# Autodesk Inventor assembly: MotorLeft
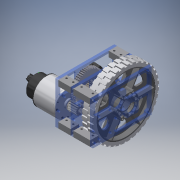
[picture p0: Inventor's stored thumbnail of the model, 180x180]
Saved by Autodesk Inventor 2019 (Build 230136000, 136)
## iProperties
Created: 2020-02-28
Part Number: MotorLeft
Document SubType Name: Assembly
Designer: james
Author: james
## Documents named in this file (13)
- F:\JimsRobot\FIRSTRobots\Design\TornadoPlatypus\MotorLeft.iam
- F:\JimsRobot\FIRSTRobots\Design\TornadoPlatypus\InsideMotorPlate.ipt
- F:\JimsRobot\FIRSTRobots\Design\Library\CTR\Falcon\217-6515 20191025.iam
- F:\JimsRobot\FIRSTRobots\Design\Library\CTR\Falcon\14T_20DP_FALCON.ipt
- F:\JimsRobot\FIRSTRobots\Design\Library\AndyMark\FR6ZZ Bearing.ipt
- F:\JimsRobot\FIRSTRobots\Design\TornadoPlatypus\MotorSpacerBlock.ipt
- F:\JimsRobot\FIRSTRobots\Design\Library\AndyMark\Toughbox d07.ipt
- F:\JimsRobot\FIRSTRobots\Design\Library\AndyMark\Toughbox d05.ipt
- F:\JimsRobot\FIRSTRobots\Design\Library\AndyMark\16t 20dp 375h with teeth.ipt
- F:\JimsRobot\FIRSTRobots\Design\Library\AndyMark\48t 20dp 500h with teeth.ipt
- F:\JimsRobot\FIRSTRobots\Design\Library\USDigital\E3-X-188-X-H-D-X.ipt
- F:\JimsRobot\FIRSTRobots\Design\Library\AndyMark\6 HiGrip Asm Rev II.iam
- F:\JimsRobot\FIRSTRobots\Design\TornadoPlatypus\MotorSpacerBlock2.ipt
## Components (19 placed, 12 different names)
1. InsideMotorPlate:1 — Mate:1, Mate:2, Mate:3, Mate:5, Mate:6, Mate:7, Mate:8, Mate:9, Mate:10, Mate:11, Flush:1, Mate:12, Flush:2, Mate:13, Flush:3, Mate:14, Flush:4, Mate:21, Mate:22, Mate:24
2. 217-6515 20191025:1 [sub-assembly] — Mate:1, Mate:2, Mate:3, Mate:4
3. 14T_20DP_FALCON:1 — Mate:4
4. FR6ZZ Bearing:1 — Mate:5, Mate:6, Mate:15, Flush:5, Mate:17
5. MotorSpacerBlock:1 — Mate:9, Mate:13, Flush:3, Mate:26, Mate:28
6. MotorSpacerBlock:2 — Mate:7, Mate:12, Flush:2
7. MotorSpacerBlock:3 — Mate:10, Mate:11, Flush:1
8. MotorSpacerBlock:4 — Mate:8, Mate:14, Flush:4, Mate:27
9. Toughbox d07:1 — Mate:15, Flush:5, Mate:16, Mate:19
10. Toughbox d05:1 — Mate:16, Mate:17, Mate:18, Mate:20
11. 16t 20dp 375h with teeth:1 — Mate:18, Mate:19
12. 48t 20dp 500h with teeth:1 — Mate:20, Mate:23
13. FR6ZZ Bearing:2 — Mate:21, Mate:22, Mate:23, Mate:25
14. E3-X-188-X-H-D-X:1 — Mate:24, Mate:25
15. InsideMotorPlate:2 — Mate:26, Mate:27, Mate:28, Mate:29, Mate:30, Mate:31, Mate:32, Mate:33, Flush:6, Mate:34, Flush:7
16. 6 HiGrip Asm Rev II:1 [sub-assembly] — Mate:29, Mate:30
17. MotorSpacerBlock2:1 — Mate:32, Mate:34, Flush:7, Mate:35, Mate:37
18. MotorSpacerBlock2:2 — Mate:31, Mate:33, Flush:6, Mate:36
19. InsideMotorPlate:3 — Mate:35, Mate:36, Mate:37
## Relationships (44: Mate 37, Flush 7)
- Mate:1: InsideMotorPlate:1 ↔ 217-6515 20191025:1
- Mate:2: InsideMotorPlate:1 ↔ 217-6515 20191025:1
- Mate:3: InsideMotorPlate:1 ↔ 217-6515 20191025:1
- Mate:4: 217-6515 20191025:1 ↔ 14T_20DP_FALCON:1
- Mate:5: InsideMotorPlate:1 ↔ FR6ZZ Bearing:1
- Mate:6: InsideMotorPlate:1 ↔ FR6ZZ Bearing:1
- Mate:7: InsideMotorPlate:1 ↔ MotorSpacerBlock:2
- Mate:8: InsideMotorPlate:1 ↔ MotorSpacerBlock:4
- Mate:9: InsideMotorPlate:1 ↔ MotorSpacerBlock:1
- Mate:10: InsideMotorPlate:1 ↔ MotorSpacerBlock:3
- Mate:11: InsideMotorPlate:1 ↔ MotorSpacerBlock:3
- Flush:1: InsideMotorPlate:1 ↔ MotorSpacerBlock:3
- Mate:12: InsideMotorPlate:1 ↔ MotorSpacerBlock:2
- Flush:2: InsideMotorPlate:1 ↔ MotorSpacerBlock:2
- Mate:13: InsideMotorPlate:1 ↔ MotorSpacerBlock:1
- Flush:3: InsideMotorPlate:1 ↔ MotorSpacerBlock:1
- Mate:14: InsideMotorPlate:1 ↔ MotorSpacerBlock:4
- Flush:4: InsideMotorPlate:1 ↔ MotorSpacerBlock:4
- Mate:15: FR6ZZ Bearing:1 ↔ Toughbox d07:1
- Flush:5: FR6ZZ Bearing:1 ↔ Toughbox d07:1
- Mate:16: Toughbox d07:1 ↔ Toughbox d05:1
- Mate:17: FR6ZZ Bearing:1 ↔ Toughbox d05:1
- Mate:18: Toughbox d05:1 ↔ 16t 20dp 375h with teeth:1
- Mate:19: Toughbox d07:1 ↔ 16t 20dp 375h with teeth:1
- Mate:20: Toughbox d05:1 ↔ 48t 20dp 500h with teeth:1
- Mate:21: InsideMotorPlate:1 ↔ FR6ZZ Bearing:2
- Mate:22: InsideMotorPlate:1 ↔ FR6ZZ Bearing:2
- Mate:23: 48t 20dp 500h with teeth:1 ↔ FR6ZZ Bearing:2
- Mate:24: InsideMotorPlate:1 ↔ E3-X-188-X-H-D-X:1
- Mate:25: FR6ZZ Bearing:2 ↔ E3-X-188-X-H-D-X:1
- Mate:26: MotorSpacerBlock:1 ↔ InsideMotorPlate:2
- Mate:27: MotorSpacerBlock:4 ↔ InsideMotorPlate:2
- Mate:28: MotorSpacerBlock:1 ↔ InsideMotorPlate:2
- Mate:29: InsideMotorPlate:2 ↔ 6 HiGrip Asm Rev II:1
- Mate:30: InsideMotorPlate:2 ↔ 6 HiGrip Asm Rev II:1
- Mate:31: InsideMotorPlate:2 ↔ MotorSpacerBlock2:2
- Mate:32: InsideMotorPlate:2 ↔ MotorSpacerBlock2:1
- Mate:33: InsideMotorPlate:2 ↔ MotorSpacerBlock2:2
- Flush:6: InsideMotorPlate:2 ↔ MotorSpacerBlock2:2
- Mate:34: InsideMotorPlate:2 ↔ MotorSpacerBlock2:1
- Flush:7: InsideMotorPlate:2 ↔ MotorSpacerBlock2:1
- Mate:35: MotorSpacerBlock2:1 ↔ InsideMotorPlate:3
- Mate:36: MotorSpacerBlock2:2 ↔ InsideMotorPlate:3
- Mate:37: MotorSpacerBlock2:1 ↔ InsideMotorPlate:3
